# Autodesk Inventor assembly: BucketR
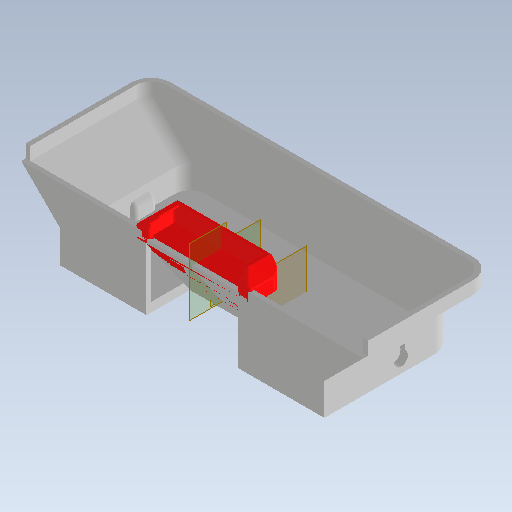
[picture p0: Inventor's stored thumbnail of the model, 512x512]
Saved by Autodesk Inventor 2022.1 (Build 261234020, 234B)
## iProperties
Created: 2022-07-23
Part Number: BucketR
Document SubType Name: Assembly
Designer: Rama
Author: Rama
## Documents named in this file (3)
- C:\Users\Rama\Desktop\GitHub\Voron-2-Mods\Mandalaroseworks\BedPan\CAD\SRC\Bucket\Bucket_SRC\Bucket_SRC_1.iam
- C:\Users\Rama\Desktop\GitHub\Voron-2-Mods\Mandalaroseworks\BedPan\CAD\SRC\Bucket\Bucket_SRC\Bucket_SRC_2.ipt
- C:\Users\Rama\Desktop\RAMA_SBNG\BedPan\Purge_Bucket\Brush_Holder.ipt
## Components (2 placed, 2 different names)
1. Bucket_Rama:1 — Passend:1, Passend:2, Passend:3, Fluchtend:1, Passend:4, Fluchtend:2
2. Brush_Holder:1 — Passend:1, Passend:4, Fluchtend:2
## Relationships (6: Mate 4, Flush 2)
- Passend:1 [Mate] (-26.8 mm): Bucket_Rama:1 ↔ Brush_Holder:1
- Passend:2 [Mate]: Bucket_Rama:1
- Passend:3 [Mate]: Bucket_Rama:1
- Fluchtend:1 [Flush] (-20 mm): Bucket_Rama:1
- Passend:4 [Mate] (10 mm): Bucket_Rama:1 ↔ Brush_Holder:1
- Fluchtend:2 [Flush]: Bucket_Rama:1 ↔ Brush_Holder:1
